# Autodesk Inventor assembly: Robot
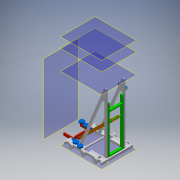
[picture p0: Inventor's stored thumbnail of the model, 180x180]
Saved by Autodesk Inventor 2016 (Build 200138000, 138)
## iProperties
Created: 2018-01-19
Part Number: Robot
Document SubType Name: Assembly
Designer: New User
Author: New User
## Documents named in this file (6)
- C:\Users\New User\Documents\Creations\2018\RobotV.2\Robot.iam
- C:\Users\New User\Documents\Creations\2018\RobotV.2\base.ipt
- C:\Users\New User\Documents\Creations\2018\RobotV.2\stage.ipt
- C:\Users\New User\Documents\Creations\2018\RobotV.2\arm.ipt
- C:\Users\New User\Documents\Creations\2018\RobotV.2\hand.ipt
- C:\Users\New User\Documents\Creations\2018\RobotV.2\wheels.ipt
## Components (6 placed, 5 different names)
1. base:1 — Mate:1, Flush:1, Mate:2, Flush:2, Angle:1, Flush:3, Mate:7, Mate:8, Mate:9, Mate:10, Mate:11, Flush:7
2. stage:1 — Mate:1, Flush:1, Mate:2, Mate:3, Mate:4
3. arm:1 — Mate:3, Mate:4, Mate:5, Mate:6
4. hand:1 — Mate:5, Mate:6, Angle:1, Mate:11, Flush:7
5. wheels:1 — Mate:7, Mate:9
6. wheels:2 — Mate:8, Mate:10
## Relationships (19: Mate 11, Flush 7, Angle 1)
- Mate:1 (12.7 mm): base:1 ↔ stage:1
- Flush:1: base:1 ↔ stage:1
- Mate:2: base:1 ↔ stage:1
- Mate:3: stage:1 ↔ arm:1
- Mate:4 (63.5 mm): stage:1 ↔ arm:1
- Mate:5: arm:1 ↔ hand:1
- Mate:6: arm:1 ↔ hand:1
- Flush:2 (406.4 mm): base:1
- Angle:1 (0 deg): base:1 ↔ hand:1
- Flush:3 (33.02 mm): base:1
- Flush:4 (-1397 mm)
- Flush:5 (-1828.8 mm)
- Mate:7: base:1 ↔ wheels:1
- Mate:8: base:1 ↔ wheels:2
- Mate:9: base:1 ↔ wheels:1
- Mate:10: base:1 ↔ wheels:2
- Mate:11: base:1 ↔ hand:1
- Flush:6 (-2044.7 mm)
- Flush:7: base:1 ↔ hand:1
